# Autodesk Inventor assembly: bl_tube_ass_2
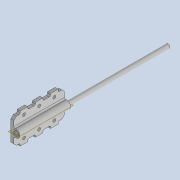
[picture p0: Inventor's stored thumbnail of the model, 180x180]
Saved by Autodesk Inventor 2020 (Build 240168000, 168)
## iProperties
Created: 2021-10-07
Part Number: bl_tube_ass_2
Document SubType Name: Assembly
Designer: Shuang Peng
Author: Shuang Peng
## Documents named in this file (3)
- D:\projects-3\torque fb tip\hardware\tip_3\bl_tube_ass_2.iam
- D:\projects-3\torque fb tip\hardware\tip_3\bw_tube_0.8_1.6.ipt
- D:\projects-3\torque fb tip\hardware\tip_3\bl_tube_hn_1.ipt
## Components (2 placed, 2 different names)
1. bw_tube_0.8_1.6:1 — Flush:1
2. bl_tube_hn_1:1 — Flush:1
## Relationships (1: Flush 1)
- Flush:1: bw_tube_0.8_1.6:1 ↔ bl_tube_hn_1:1
